# Autodesk Inventor assembly: AssemblyUflow
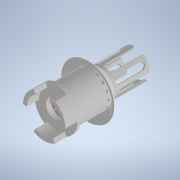
[picture p0: Inventor's stored thumbnail of the model, 180x180]
Saved by Autodesk Inventor 2022.4 (Build 264492010, 492A)
## iProperties
Created: 2023-09-20
Part Number: AssemblyUflow
Document SubType Name: Assembly
Designer: tmass
Author: tmass
## Documents named in this file (6)
- C:\Users\tmass\OneDrive\Bureau\UFO paper\3D models\Uflow\Inventor\AssemblyUflow.iam
- C:\Users\tmass\OneDrive\Bureau\UFO paper\3D models\Uflow\Inventor\Box.ipt
- C:\Users\tmass\OneDrive\Bureau\UFO paper\3D models\Uflow\Inventor\Top cover.ipt
- C:\Users\tmass\OneDrive\Bureau\UFO paper\3D models\Uflow\Inventor\Reflector+feet.ipt
- C:\Users\tmass\OneDrive\Bureau\UFO paper\3D models\Uflow\Inventor\Top holder magnet.ipt
- C:\Users\tmass\OneDrive\Bureau\UFO paper\3D models\Uflow\Inventor\holder no magnet.ipt
## Components (5 placed, 5 different names)
1. Box:1 — Mate:8, Mate:9, Mate:11
2. Top cover:1 — Mate:5, Mate:6, Mate:7, Mate:8, Mate:9, Mate:10
3. Reflector+feet:1 — Mate:10, Mate:11
4. Top holder magnet:1 — Mate:3, Mate:4, Mate:5, Mate:6
5. holder no magnet:1 — Mate:3, Mate:4, Mate:7
## Relationships (9: Mate 9)
- Mate:3: Top holder magnet:1 ↔ holder no magnet:1
- Mate:4: Top holder magnet:1 ↔ holder no magnet:1
- Mate:5: Top cover:1 ↔ Top holder magnet:1
- Mate:6: Top cover:1 ↔ Top holder magnet:1
- Mate:7: Top cover:1 ↔ holder no magnet:1
- Mate:8: Box:1 ↔ Top cover:1
- Mate:9: Box:1 ↔ Top cover:1
- Mate:10: Top cover:1 ↔ Reflector+feet:1
- Mate:11: Box:1 ↔ Reflector+feet:1
